# Autodesk Inventor assembly: Locking Pin Assy
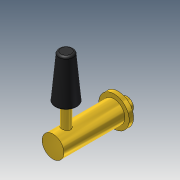
[picture p0: Inventor's stored thumbnail of the model, 180x180]
Saved by Autodesk Inventor 2011 (Build 150239000, 239)
## iProperties
Created: 2012-11-06
Part Number: Locking Pin Assy
Document SubType Name: Assembly
Designer: Lance
Author: Lance
## Documents named in this file (4)
- C:\Inventor Projects\MPX0032 - Projector Accessories\Manfrotto 494RC2 - Tripod Head\Locking Pin Assy.iam
- C:\Inventor Projects\MPX0032 - Projector Accessories\Manfrotto 494RC2 - Tripod Head\Locking Pin.ipt
- C:\Inventor Projects\MPX0032 - Projector Accessories\Manfrotto 494RC2 - Tripod Head\Locking Pin Lever.ipt
- C:\Inventor Projects\MPX0032 - Projector Accessories\Manfrotto 494RC2 - Tripod Head\Locking Pin Lever Rubber.ipt
## Components (3 placed, 3 different names)
1. Locking Pin:1 — Mate:1, Tangent:1, Flush:1
2. Locking Pin Lever:1 — Mate:1, Tangent:1, Flush:1, Insert:1, Flush:2
3. Locking Pin Lever Rubber:1 — Insert:1, Flush:2
## Relationships (5: Flush 2, Mate 1, Tangent 1, Insert 1)
- Mate:1: Locking Pin:1 ↔ Locking Pin Lever:1
- Tangent:1: Locking Pin:1 ↔ Locking Pin Lever:1
- Flush:1: Locking Pin:1 ↔ Locking Pin Lever:1
- Insert:1: Locking Pin Lever:1 ↔ Locking Pin Lever Rubber:1
- Flush:2: Locking Pin Lever:1 ↔ Locking Pin Lever Rubber:1
